# Autodesk Inventor assembly: Assem1
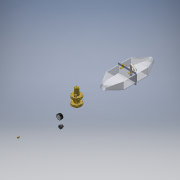
[picture p0: Inventor's stored thumbnail of the model, 180x180]
Saved by Autodesk Inventor 2017 (Build 210142000, 142)
## iProperties
Created: 2014-08-02
Part Number: Assem1
Document SubType Name: Assembly
Designer: XuZhiqing
Sending System: SolidWorks 2014
Last Author: 1
Last Saved: 2014-09-23
Author: XuZhiqing
## Documents named in this file (16)
- C:\Users\XuZhiqing\Desktop\Project01-CFD_the_sys\CAD-Whole Sys\filter and gauge\gas pressure gauge\gas pressure gauge.iam
- C:\Users\XuZhiqing\Desktop\Project01-CFD_the_sys\CAD-Whole Sys\filter and gauge\gas pressure gauge\Part4.ipt
- C:\Users\XuZhiqing\Desktop\Project01-CFD_the_sys\CAD-Whole Sys\filter and gauge\gas pressure gauge\Part6.ipt
- C:\Users\XuZhiqing\Desktop\Project01-CFD_the_sys\CAD-Whole Sys\filter and gauge\gas pressure gauge\Part5.ipt
- C:\Users\XuZhiqing\Desktop\Project01-CFD_the_sys\CAD-Whole Sys\filter and gauge\gas pressure gauge\Part7.ipt
- C:\Users\XuZhiqing\Desktop\Project01-CFD_the_sys\CAD-Whole Sys\filter and gauge\gas pressure gauge\Part8.ipt
- C:\Users\XuZhiqing\Desktop\Project01-CFD_the_sys\CAD-Whole Sys\filter and gauge\gas pressure gauge\Part10.ipt
- C:\Users\XuZhiqing\Desktop\Project01-CFD_the_sys\CAD-Whole Sys\filter and gauge\gas pressure gauge\Part12.ipt
- C:\Users\XuZhiqing\Desktop\Project01-CFD_the_sys\CAD-Whole Sys\filter and gauge\gas pressure gauge\Part17.ipt
- C:\Users\XuZhiqing\Desktop\Project01-CFD_the_sys\CAD-Whole Sys\filter and gauge\gas pressure gauge\Part19.ipt
- C:\Users\XuZhiqing\Desktop\Project01-CFD_the_sys\CAD-Whole Sys\filter and gauge\gas pressure gauge\socket head cap screw_am.ipt
- C:\Users\XuZhiqing\Desktop\Project01-CFD_the_sys\CAD-Whole Sys\filter and gauge\gas pressure gauge\Part21.ipt
- C:\Users\XuZhiqing\Desktop\Project01-CFD_the_sys\CAD-Whole Sys\filter and gauge\gas pressure gauge\Solid5.ipt
- C:\Users\XuZhiqing\Desktop\Project01-CFD_the_sys\CAD-Whole Sys\filter and gauge\gas pressure gauge\gauge3.ipt
- C:\Users\XuZhiqing\Desktop\Project01-CFD_the_sys\CAD-Whole Sys\filter and gauge\gas pressure gauge\Solid9.ipt
- C:\Users\XuZhiqing\Desktop\Project01-CFD_the_sys\CAD-Whole Sys\filter and gauge\filter\Assem1.iam
## Components (26 placed, 15 different names)
1. Part4:1
2. Part6:1
3. Part5:2
4. Part7:1
5. Part8:1
6. Part10:1 — Mate:2, Mate:3, Mate:4, Mate:5
7. Part12:1
8. Part17:1
9. Part19:1 — Mate:4, Mate:5
10. socket head cap screw_am:26
11. socket head cap screw_am:27
12. socket head cap screw_am:28
13. socket head cap screw_am:29
14. socket head cap screw_am:30
15. socket head cap screw_am:31
16. socket head cap screw_am:32
17. socket head cap screw_am:33
18. socket head cap screw_am:34
19. socket head cap screw_am:36
20. socket head cap screw_am:37
21. socket head cap screw_am:38
22. Part21:1 — Mate:1, Mate:2, Mate:3
23. Solid5:1
24. gauge3:1
25. Solid9:1
26. Assem1:1 [sub-assembly] — Mate:1
## Relationships (5: Mate 5)
- Mate:1: Part21:1 ↔ Assem1:1
- Mate:2: Part10:1 ↔ Part21:1
- Mate:3: Part10:1 ↔ Part21:1
- Mate:4: Part10:1 ↔ Part19:1
- Mate:5: Part10:1 ↔ Part19:1
